# Autodesk Inventor assembly: Navi versie 2
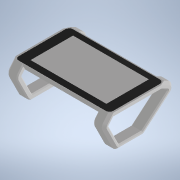
[picture p0: Inventor's stored thumbnail of the model, 180x180]
Saved by Autodesk Inventor 2022 (Build 260153000, 153)
## iProperties
Created: 2021-09-21
Part Number: Navi versie 2
Document SubType Name: Assembly
Designer: Frank
Author: Frank
## Documents named in this file (7)
- C:\Users\Frank\OneDrive\Documents\Inventor\Yamaha XTZ 750\Navisystem 2\Rollbar screen mount raspberry pi.iam
- C:\Users\Frank\OneDrive\Documents\Inventor\Yamaha XTZ 750\Navisystem 2\Rollbar main body.ipt
- C:\Users\Frank\OneDrive\Documents\Inventor\Yamaha XTZ 750\Navisystem 2\Raspberry touchscreen.ipt
- C:\Users\Frank\OneDrive\Documents\Inventor\Yamaha XTZ 750\Navisys\raspberry-pi-4-model-b-1.snapshot.3\Raspberry Pi 4 Model B.ipt
- C:\Users\Frank\OneDrive\Documents\Inventor\Yamaha XTZ 750\Navisystem 2\Rollbar left body.ipt
- C:\Users\Frank\OneDrive\Documents\Inventor\Yamaha XTZ 750\Navisystem 2\Rollbar right body.ipt
- C:\Users\Frank\OneDrive\Documents\Inventor\Yamaha XTZ 750\Navisystem 2\Rollbar base plate.ipt
## Components (6 placed, 6 different names)
1. Rollbar main body:1 — Mate:2, Mate:3
2. Rollbar left body:1 — Mate:8, Mate:9
3. Rollbar right body:1 — Flush:1, Mate:7
4. Rollbar base plate:1 — Mate:7, Mate:8, Mate:9
5. Raspberry touchscreen:1 — Mate:2, Mate:3, Mate:4, Mate:5, Mate:6, Flush:1
6. Raspberry Pi 4 Model B:1 — Mate:4, Mate:5, Mate:6
## Relationships (9: Mate 8, Flush 1)
- Mate:2: Rollbar main body:1 ↔ Raspberry touchscreen:1
- Mate:3: Rollbar main body:1 ↔ Raspberry touchscreen:1
- Mate:4: Raspberry touchscreen:1 ↔ Raspberry Pi 4 Model B:1
- Mate:5: Raspberry touchscreen:1 ↔ Raspberry Pi 4 Model B:1
- Mate:6: Raspberry touchscreen:1 ↔ Raspberry Pi 4 Model B:1
- Flush:1: Rollbar right body:1 ↔ Raspberry touchscreen:1
- Mate:7: Rollbar right body:1 ↔ Rollbar base plate:1
- Mate:8: Rollbar left body:1 ↔ Rollbar base plate:1
- Mate:9: Rollbar left body:1 ↔ Rollbar base plate:1
